# Autodesk Inventor assembly: User Library-OLED-1_3-128X64
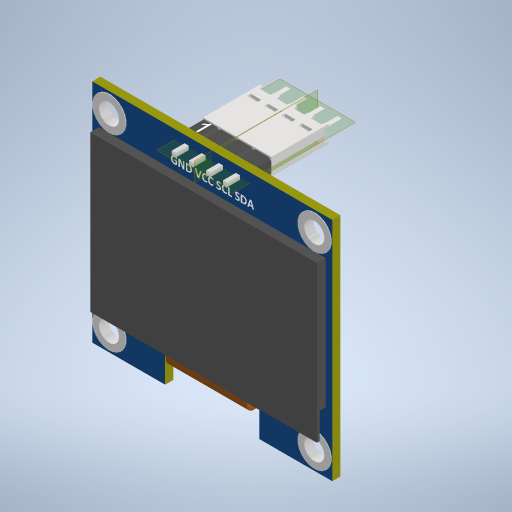
[picture p0: Inventor's stored thumbnail of the model, 512x512]
Saved by Autodesk Inventor 2024.3 (Build 283343000, 343)
## iProperties
Created: 2021-07-30
Part Number: User Library-OLED-1_3-128X64
Document SubType Name: Assembly
Designer: Yann
Sending System: SOLIDWORKS 2021-2020322
MC: AMD64
MC_MODEL: Intel64 Family 6 Model 58 Stepping 0, GenuineIntel
OS: Windows_NT
FRU: Parasolid Version 32.1, build 251,  9-25-2020
FORMAT: text
GUISE: transmit
FILE: 14F0D745-A58B-49F1-9959-010D867F6CC6.x_t
DATE: Fri Jul 30 19:00:30 2021
Author: Yann
## Documents named in this file (5)
- C:\Users\atrus\Dropbox\elec\Mechanical\DCBuddyV2\User Library-OLED-1_3-128X64.iam
- C:\Users\atrus\Dropbox\elec\Mechanical\DCBuddyV2\User Library-OLED-1_3-128X64.ipt
- C:\Users\atrus\Dropbox\elec\Mechanical\DCBuddyV2\User Library-OLED-1_3-128X64_1.ipt
- C:\Users\atrus\Dropbox\elec\Mechanical\DCBuddyV2\User Library-OLED-1_3-128X64_2.ipt
- C:\Users\atrus\Dropbox\elec\Mechanical\DCBuddyV2\901471104.ipt
## Components (4 placed, 4 different names)
1. User Library-OLED-1_3-128X64
2. User Library-OLED-1_3-128X64_1
3. User Library-OLED-1_3-128X64_2 — Mate:1, Flush:1, Flush:2
4. 901471104:1 — Mate:1, Flush:1, Flush:2
## Relationships (3: Flush 2, Mate 1)
- Mate:1: User Library-OLED-1_3-128X64_2 ↔ 901471104:1
- Flush:1: User Library-OLED-1_3-128X64_2 ↔ 901471104:1
- Flush:2: User Library-OLED-1_3-128X64_2 ↔ 901471104:1
